# Autodesk Inventor assembly: 2016-02-05-RhinoRobotV09
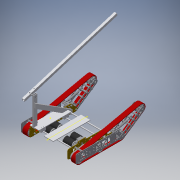
[picture p0: Inventor's stored thumbnail of the model, 180x180]
Saved by Autodesk Inventor 2016 SP1 (Build 200210100, 210)
## iProperties
Created: 2016-01-23
Part Number: 2016-02-05-RhinoRobotV09
Document SubType Name: Assembly
Designer: steele
Mass: 23360.3 g
Surface Area: 43274.3 cm^2
Volume: 23034.6 cm^3
Density: 1.01414 g/cm^3
Author: steele
## Documents named in this file (12)
- C:\snobotics\CAD-Development\robSteele\SnoBotics2016\2015-02-05-RhinoRobotNarrowView\2016-02-05-RhinoRobotV09.iam
- C:\snobotics\CAD-Development\robSteele\SnoBotics2016\RhinoTrackDriveModule\am-3322+RhinoTrackDriveModule.iam
- C:\snobotics\CAD-Development\robSteele\SnoBotics2016\RhinoBottomFloorOptions\RhinoBottomFloorPlate01.ipt
- C:\snobotics\CAD-Development\robSteele\SnoBotics2016\RhinoTrackDriveModule\am-3322+RhinoTrackDriveModule_MIR9.iam
- C:\snobotics\CAD-Development\robSteele\SnoBotics2016\2016-01-31-Lift\2016-01-31-LiftTiltAssembly.iam
- C:\snobotics\CAD-Development\robSteele\SnoBotics2016\AM Parts\Churo_16_5_inches.ipt
- C:\snobotics\CAD-Development\robSteele\SnoBotics2016\2016-01-31-Lift\longSupportPlate.ipt
- C:\snobotics\CAD-Development\robSteele\SnoBotics2016\2016-01-31-Lift\shortSupportPlate.ipt
- C:\snobotics\CAD-Development\robSteele\SnoBotics2016\2016-01-31-Lift\U_bolt.ipt
- C:\snobotics\CAD-Development\robSteele\SnoBotics2016\2016-01-31-Lift\LiftSpacer.ipt
- C:\snobotics\CAD-Development\robSteele\SnoBotics2016\TelescopeArm\OuterTube.ipt
- C:\snobotics\CAD-Development\robSteele\SnoBotics2016\2016-01-31-Lift\shortAxel.ipt
## Components (13 placed, 11 different names)
1. RhinoBottomFloorPlate01:1 — Mate:1, Flush:2, Flush:11, Flush:14, Mate:18, Flush:15
2. am-3322+RhinoTrackDriveModule:1 [sub-assembly] — Mate:1, Flush:2, Flush:11, Insert:1, Insert:2, Insert:6, Flush:16, Mate:19, Mate:20, Flush:19, Mate:22
3. am-3322+RhinoTrackDriveModule_MIR9:1 [sub-assembly]
4. 2016-01-31-LiftTiltAssembly:1 [sub-assembly] — Flush:14, Mate:18, Flush:15
5. Churo_16_5_inches:1 — Insert:1, Tangent:1, Flush:18, Tangent:3, Tangent:4
6. Churo_16_5_inches:2 — Insert:2
7. Churo_16_5_inches:6 — Insert:6, Tangent:2
8. longSupportPlate:1 — Tangent:1, Tangent:2, Flush:16, Flush:17
9. shortSupportPlate:1 — Mate:21, Flush:19, Mate:22, Insert:8
10. U_bolt:1 — Tangent:3, Mate:19
11. LiftSpacer:1 — Tangent:4, Mate:20, Mate:21
12. OuterTube:1 — Insert:7
13. shortAxel:1 — Insert:7, Insert:8
## Relationships (23: Flush 8, Mate 6, Insert 5, Tangent 4)
- Mate:1: RhinoBottomFloorPlate01:1 ↔ am-3322+RhinoTrackDriveModule:1
- Flush:2: RhinoBottomFloorPlate01:1 ↔ am-3322+RhinoTrackDriveModule:1
- Flush:11: RhinoBottomFloorPlate01:1 ↔ am-3322+RhinoTrackDriveModule:1
- Flush:14: RhinoBottomFloorPlate01:1 ↔ 2016-01-31-LiftTiltAssembly:1
- Mate:18: RhinoBottomFloorPlate01:1 ↔ 2016-01-31-LiftTiltAssembly:1
- Flush:15: RhinoBottomFloorPlate01:1 ↔ 2016-01-31-LiftTiltAssembly:1
- Insert:1: am-3322+RhinoTrackDriveModule:1 ↔ Churo_16_5_inches:1
- Insert:2: am-3322+RhinoTrackDriveModule:1 ↔ Churo_16_5_inches:2
- Insert:6: am-3322+RhinoTrackDriveModule:1 ↔ Churo_16_5_inches:6
- Tangent:1: Churo_16_5_inches:1 ↔ longSupportPlate:1
- Tangent:2: Churo_16_5_inches:6 ↔ longSupportPlate:1
- Flush:16: am-3322+RhinoTrackDriveModule:1 ↔ longSupportPlate:1
- Flush:17: longSupportPlate:1
- Flush:18: Churo_16_5_inches:1
- Tangent:3: Churo_16_5_inches:1 ↔ U_bolt:1
- Mate:19 (12.7 mm): am-3322+RhinoTrackDriveModule:1 ↔ U_bolt:1
- Tangent:4: Churo_16_5_inches:1 ↔ LiftSpacer:1
- Mate:20: am-3322+RhinoTrackDriveModule:1 ↔ LiftSpacer:1
- Mate:21: shortSupportPlate:1 ↔ LiftSpacer:1
- Flush:19: am-3322+RhinoTrackDriveModule:1 ↔ shortSupportPlate:1
- Mate:22: am-3322+RhinoTrackDriveModule:1 ↔ shortSupportPlate:1
- Insert:7: OuterTube:1 ↔ shortAxel:1
- Insert:8: shortSupportPlate:1 ↔ shortAxel:1
## Named parameters: robotWidth = 660.4 mm, halfRobotWidth = 330.2 mm, maxPerimeter = 3048 mm, maxLength = 863.6 mm, widthOfTrack = 95.25 mm, boardWidth = 469.9 mm
